# Autodesk Inventor assembly: Second Base Extension (Draft 2)
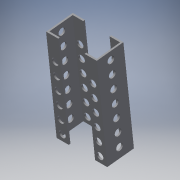
[picture p0: Inventor's stored thumbnail of the model, 180x180]
Saved by Autodesk Inventor 2018 (Build 220112000, 112)
## iProperties
Created: 2017-06-28
Part Number: Second Base Extension (Draft 2)
Document SubType Name: Assembly
Designer: James
Author: James
## Documents named in this file (4)
- C:\Users\James\Desktop\EE REU\Hardware\Vex Arm\Vex Arm Draft 2\Second Base Extension (Draft 2).iam
- C:\Users\James\Desktop\EE REU\Hardware\Vex Arm\Vex Parts\Base C Channel.ipt
- C:\Users\James\Desktop\EE REU\Hardware\Vex Arm\Vex Parts\393motor.ipt
- C:\Users\James\Desktop\EE REU\Hardware\Vex Arm\Vex Parts\Vex Potentiometer.ipt
## Components (4 placed, 3 different names)
1. Base C Channel:1 — Mate:1, Flush:1, Flush:2, Insert:1
2. Base C Channel:2 — Mate:1, Flush:1, Flush:2, Insert:2
3. 393motor:1 — Insert:1
4. Vex Potentiometer:1 — Insert:2
## Relationships (5: Flush 2, Insert 2, Mate 1)
- Mate:1 (45 mm): Base C Channel:1 ↔ Base C Channel:2
- Flush:1: Base C Channel:1 ↔ Base C Channel:2
- Flush:2: Base C Channel:1 ↔ Base C Channel:2
- Insert:1: Base C Channel:1 ↔ 393motor:1
- Insert:2: Base C Channel:2 ↔ Vex Potentiometer:1
